# Autodesk Inventor assembly: GP5-100-TAV
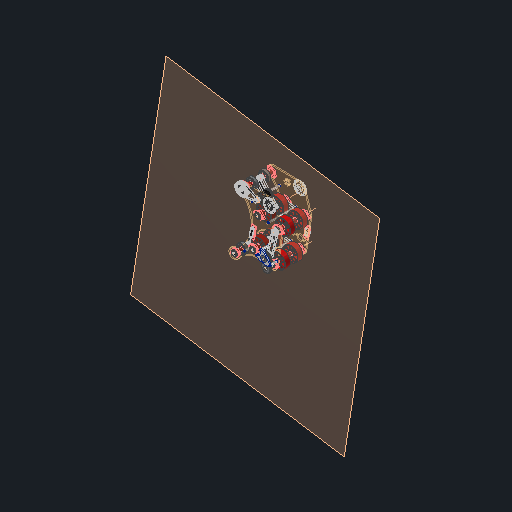
[picture p0: Inventor's stored thumbnail of the model, 512x512]
Saved by Autodesk Inventor 2023.4 (Build 274418000, 418)
## iProperties
Created: 2025-02-03
Part Number: GP5-100-TAV
Document SubType Name: Assembly
Designer: slick
Mass: 3623.08 g
Surface Area: 8652.96 cm^2
Volume: 1639.13 cm^3
Density: 2.21037 g/cm^3
Author: slick
## Documents named in this file (32)
- C:\Users\brand\OneDrive\Documents\GitHub\robotics 23\2025-ReefScape---CAD\Gripper\GP5\GP5-100-TAV.iam
- C:\Users\brand\OneDrive\Documents\GitHub\robotics 23\2025-ReefScape---CAD\Gripper\GP5\GP5-003.ipt
- C:\Users\brand\OneDrive\Documents\GitHub\robotics 23\2025-ReefScape---CAD\COMMON PARTS\BEARINGS\13_75mm_1_2_ThunderHex_ID_x_1_125_OD_x_0_313_WD_Flanged_Bearing_217-4006_MIR.ipt
- C:\Users\brand\OneDrive\Documents\GitHub\robotics 23\2025-ReefScape---CAD\Gripper\GP5\GP5-005.ipt
- C:\Users\brand\OneDrive\Documents\GitHub\robotics 23\2025-ReefScape---CAD\COMMON PARTS\WHEELS\2_OD_Straight_Flex_Wheel_217-6354.ipt
- C:\Users\brand\OneDrive\Documents\GitHub\robotics 23\2025-ReefScape---CAD\COMMON PARTS\WHEELS\am-3946 3IN 375Hex Compliant Wheel REV 3.ipt
- C:\Users\brand\OneDrive\Documents\GitHub\robotics 23\2025-ReefScape---CAD\COMMON PARTS\MOTORS\Minion.ipt
- C:\Users\brand\OneDrive\Documents\GitHub\robotics 23\2025-ReefScape---CAD\COMMON PARTS\PULLEYS\gt2\16T Gt2 Kracken PullyWCP-1178.ipt
- C:\Users\brand\OneDrive\Documents\GitHub\robotics 23\2025-ReefScape---CAD\COMMON PARTS\PULLEYS\gt2\60t_x_9mm_Wide_Double_Flange_Aluminum_Pulley_GT2_3mm_1_2_Hex_Bore_217-5876.ipt
- C:\Users\brand\OneDrive\Documents\GitHub\robotics 23\2025-ReefScape---CAD\COMMON PARTS\PULLEYS\gt2\24t_x_9mm_Wide_Double_Flange_Aluminum_Pulley_GT2_3mm_1_2_Hex_Bore_217-5875.ipt
- C:\Users\brand\OneDrive\Documents\GitHub\robotics 23\2025-ReefScape---CAD\COMMON PARTS\GEARS\20dp .5 hex\34t_Aluminum_Spur_Gear_20_DP_1_2_Hex_Bore_217-2706.ipt
- C:\Users\brand\OneDrive\Documents\GitHub\robotics 23\2025-ReefScape---CAD\Gripper\GP5\GP5-007.ipt
- C:\Users\brand\OneDrive\Documents\GitHub\robotics 23\2025-ReefScape---CAD\COMMON PARTS\BEARINGS\Bearing Retainer\Retainer.ipt
- C:\Users\brand\OneDrive\Documents\GitHub\robotics 23\2025-ReefScape---CAD\Gripper\GP5\GT2-100T.ipt
- C:\Users\brand\OneDrive\Documents\GitHub\robotics 23\2025-ReefScape---CAD\Gripper\GP5\GT2-90T.ipt
- C:\Users\brand\OneDrive\Documents\GitHub\robotics 23\2025-ReefScape---CAD\Gripper\GP5\GT2-90T16-60.ipt
- C:\Users\brand\OneDrive\Documents\GitHub\robotics 23\2025-ReefScape---CAD\Gripper\GP5\GT2-105T.ipt
- C:\Users\brand\OneDrive\Documents\GitHub\robotics 23\2025-ReefScape---CAD\Gripper\GP5\GP5-014.ipt
- C:\Users\brand\OneDrive\Documents\GitHub\robotics 23\2025-ReefScape---CAD\Gripper\GP5\GP5-019.ipt
- C:\Users\brand\OneDrive\Documents\GitHub\robotics 23\2025-ReefScape---CAD\COMMON PARTS\HUBS\WCP-1388.ipt
- C:\Users\brand\OneDrive\Documents\GitHub\robotics 23\2025-ReefScape---CAD\Gripper\GP5\GP5-023.ipt
- C:\Users\brand\OneDrive\Documents\GitHub\robotics 23\2025-ReefScape---CAD\Gripper\GP5\GP5-024.ipt
- C:\Users\brand\OneDrive\Documents\GitHub\robotics 23\2025-ReefScape---CAD\Gripper\GP5\GP5-025.ipt
- C:\Users\brand\OneDrive\Documents\GitHub\robotics 23\2025-ReefScape---CAD\Gripper\GP5\GP5-026.ipt
- C:\Users\brand\OneDrive\Documents\GitHub\robotics 23\2025-ReefScape---CAD\Gripper\GP5\GP5-013.ipt
- C:\Users\brand\OneDrive\Documents\GitHub\robotics 23\2025-ReefScape---CAD\Gripper\GP5\GP5-015.ipt
- C:\Users\brand\OneDrive\Documents\GitHub\robotics 23\2025-ReefScape---CAD\Gripper\GP5\GP5-016.ipt
- C:\Users\brand\OneDrive\Documents\GitHub\robotics 23\2025-ReefScape---CAD\Gripper\GP5\GP5-027.ipt
- C:\Users\brand\OneDrive\Documents\GitHub\robotics 23\2025-ReefScape---CAD\Gripper\GP5\GP5-028.ipt
- C:\Users\brand\OneDrive\Documents\GitHub\robotics 23\2025-ReefScape---CAD\Gripper\GP5\GP5-029.ipt
- C:\Users\brand\OneDrive\Documents\GitHub\robotics 23\2025-ReefScape---CAD\COMMON PARTS\BEARINGS\0_500_ID_x_1_125_OD_x_0_313_WD_Flanged_Bearing_217-2731.ipt
- C:\Users\brand\OneDrive\Documents\GitHub\robotics 23\2025-ReefScape---CAD\STEP files\sen36005_3d_model\With Flush Mount Spacer.iam
## Components (104 placed, 31 different names)
1. Minion:1 — Mate:18, Insert:15, Mate:19, Flush:1, Mate:22
2. 34t_Aluminum_Spur_Gear_20_DP_1_2_Hex_Bore_217-2706:1 — Mate:53, Flush:16, Mate:121
3. 34t_Aluminum_Spur_Gear_20_DP_1_2_Hex_Bore_217-2706:2 — Mate:51, Flush:16, Mate:56, Mate:72, Flush:78
4. WCP-1388:1 — Mate:80, Mate:81, Insert:54
5. WCP-1388:2 — Mate:79, Mate:81, Insert:53
6. GP5-026:1 — Insert:49, Insert:50
7. GP5-026:2 — Insert:45, Insert:46
8. GP5-026:3 — Insert:47, Insert:48
9. GP5-026:4 — Insert:51, Insert:52
10. GP5-014:3 — Mate:82, Mate:83
11. GP5-014:4 — Mate:84, Mate:85
12. GP5-015:1 — Mate:86, Mate:87
13. GP5-016:1 — Mate:88, Mate:89
14. GP5-016:2 — Mate:92, Mate:93
15. GP5-015:2 — Mate:97, Mate:100
16. GP5-015:3 — Mate:96, Mate:98
17. GP5-015:4 — Mate:95, Mate:99
18. GP5-013:2 — Mate:101, Mate:102
19. GP5-019:3 — Mate:104, Mate:105
20. GP5-019:4 — Mate:103, Mate:106
21. GP5-013:4 — Mate:108, Mate:109
22. GP5-013:5 — Mate:111, Mate:117
23. GP5-013:7 — Mate:113, Mate:116
24. GP5-027:1 — Insert:60, Insert:62, Insert:63, Mate:120
25. 0_500_ID_x_1_125_OD_x_0_313_WD_Flanged_Bearing_217-2731:1 — Insert:60, Mate:119, Flush:74, Mate:121
26. GP5-028:1 — Insert:62, Insert:64
27. GP5-028:2 — Insert:63, Insert:65
28. GP5-028:3 — Insert:58
29. GP5-029:1 — Mate:119, Flush:74
30. 0_500_ID_x_1_125_OD_x_0_313_WD_Flanged_Bearing_217-2731:2 — Insert:66
31. With Flush Mount Spacer:1 [sub-assembly] — Insert:69, Insert:70
32. With Flush Mount Spacer:2 [sub-assembly] — Insert:67, Insert:68
33. Retainer:13 — Insert:24, Insert:25
34. Retainer:12 — Insert:26, Insert:27
35. Retainer:11 — Insert:34, Insert:35
36. Retainer:10 — Insert:28, Insert:29
37. Retainer:9 — Insert:32, Insert:33
38. Retainer:8 — Insert:30, Insert:31
39. Retainer:7 — Insert:16, Insert:17
40. Retainer:6 — Insert:21, Insert:22
41. Retainer:5 — Insert:20, Insert:23
42. Retainer:4 — Insert:36, Insert:37, Insert:39
43. Retainer:3 — Insert:18, Insert:19
44. Retainer:1 — Insert:38, Insert:44
45. 13_75mm_1_2_ThunderHex_ID_x_1_125_OD_x_0_313_WD_Flanged_Bearing_217-4006_MIR:6 — Insert:9, Mate:13
46. 13_75mm_1_2_ThunderHex_ID_x_1_125_OD_x_0_313_WD_Flanged_Bearing_217-4006_MIR:14 — Insert:7, Mate:16, Mate:24
47. 13_75mm_1_2_ThunderHex_ID_x_1_125_OD_x_0_313_WD_Flanged_Bearing_217-4006_MIR:13 — Insert:8, Mate:12, Mate:64, Mate:66, Mate:67, Mate:69, Flush:73
48. 13_75mm_1_2_ThunderHex_ID_x_1_125_OD_x_0_313_WD_Flanged_Bearing_217-4006_MIR:12 — Insert:2
49. 13_75mm_1_2_ThunderHex_ID_x_1_125_OD_x_0_313_WD_Flanged_Bearing_217-4006_MIR:11 — Insert:6, Flush:82
50. 13_75mm_1_2_ThunderHex_ID_x_1_125_OD_x_0_313_WD_Flanged_Bearing_217-4006_MIR:10 — Insert:3, Flush:85
51. 13_75mm_1_2_ThunderHex_ID_x_1_125_OD_x_0_313_WD_Flanged_Bearing_217-4006_MIR:9 — Insert:5, Flush:83
52. 13_75mm_1_2_ThunderHex_ID_x_1_125_OD_x_0_313_WD_Flanged_Bearing_217-4006_MIR:8 — Insert:4
53. 13_75mm_1_2_ThunderHex_ID_x_1_125_OD_x_0_313_WD_Flanged_Bearing_217-4006_MIR:7 — Insert:1, Mate:28
54. 13_75mm_1_2_ThunderHex_ID_x_1_125_OD_x_0_313_WD_Flanged_Bearing_217-4006_MIR:5 — Insert:11, Mate:17, Mate:123
55. 13_75mm_1_2_ThunderHex_ID_x_1_125_OD_x_0_313_WD_Flanged_Bearing_217-4006_MIR:4 — Insert:10, Mate:14, Mate:26
56. 13_75mm_1_2_ThunderHex_ID_x_1_125_OD_x_0_313_WD_Flanged_Bearing_217-4006_MIR:3 — Insert:12, Mate:15, Mate:20, Mate:21
57. 24t_x_9mm_Wide_Double_Flange_Aluminum_Pulley_GT2_3mm_1_2_Hex_Bore_217-5875:7 — Mate:64, Mate:65
58. 24t_x_9mm_Wide_Double_Flange_Aluminum_Pulley_GT2_3mm_1_2_Hex_Bore_217-5875:8 — Mate:46, Flush:12
59. 24t_x_9mm_Wide_Double_Flange_Aluminum_Pulley_GT2_3mm_1_2_Hex_Bore_217-5875:9 — Mate:57, Mate:58, Mate:71
60. 24t_x_9mm_Wide_Double_Flange_Aluminum_Pulley_GT2_3mm_1_2_Hex_Bore_217-5875:10 — Mate:47, Mate:78, Flush:71, Flush:81, Flush:84
61. 24t_x_9mm_Wide_Double_Flange_Aluminum_Pulley_GT2_3mm_1_2_Hex_Bore_217-5875:12 — Mate:43, Mate:44, Flush:11, Flush:65, Mate:84
62. 24t_x_9mm_Wide_Double_Flange_Aluminum_Pulley_GT2_3mm_1_2_Hex_Bore_217-5875:13 — Mate:31, Mate:32, Flush:9, Mate:37, Mate:38, Mate:41
63. 24t_x_9mm_Wide_Double_Flange_Aluminum_Pulley_GT2_3mm_1_2_Hex_Bore_217-5875:14 — Mate:33, Mate:34, Flush:10, Mate:39
64. 24t_x_9mm_Wide_Double_Flange_Aluminum_Pulley_GT2_3mm_1_2_Hex_Bore_217-5875:15 — Mate:60, Mate:62, Flush:65, Flush:66, Flush:67
65. 24t_x_9mm_Wide_Double_Flange_Aluminum_Pulley_GT2_3mm_1_2_Hex_Bore_217-5875:16 — Mate:59, Mate:61, Mate:65, Flush:68
66. GT2-90T16-60:1 — Mate:22, Mate:23, Flush:2
67. GT2-105T:1 — Mate:52, Mate:54, Flush:77
68. GT2-100T:5 — Mate:69, Mate:70, Flush:68
69. GT2-90T:2 — Mate:71, Mate:72, Mate:73
70. GT2-90T:1 — Mate:77, Mate:78, Flush:71
71. GT2-100T:3 — Mate:67, Mate:68, Flush:67
72. GT2-100T:2 — Mate:36, Flush:10, Mate:44, Flush:11
73. GT2-100T:1 — Mate:35, Flush:9, Mate:45, Flush:12
74. 16T Gt2 Kracken PullyWCP-1178:1 — Mate:19, Flush:1
75. 60t_x_9mm_Wide_Double_Flange_Aluminum_Pulley_GT2_3mm_1_2_Hex_Bore_217-5876:1 — Mate:20, Mate:21, Mate:23, Flush:2, Flush:3
76. 24t_x_9mm_Wide_Double_Flange_Aluminum_Pulley_GT2_3mm_1_2_Hex_Bore_217-5875:1 — Mate:52, Mate:53, Flush:79, Mate:120
77. 24t_x_9mm_Wide_Double_Flange_Aluminum_Pulley_GT2_3mm_1_2_Hex_Bore_217-5875:2 — Mate:66, Flush:66, Mate:82
78. 24t_x_9mm_Wide_Double_Flange_Aluminum_Pulley_GT2_3mm_1_2_Hex_Bore_217-5875:4 — Mate:76, Mate:77, Flush:77, Flush:79, Mate:123
79. 24t_x_9mm_Wide_Double_Flange_Aluminum_Pulley_GT2_3mm_1_2_Hex_Bore_217-5875:5 — Mate:49, Flush:81, Mate:122
80. 24t_x_9mm_Wide_Double_Flange_Aluminum_Pulley_GT2_3mm_1_2_Hex_Bore_217-5875:6 — Mate:56, Mate:58, Mate:73, Flush:84
81. GP5-014:1 — Mate:32, Mate:33, Mate:35, Mate:36, Mate:38, Mate:39
82. GP5-014:2 — Mate:59, Mate:60, Mate:61, Mate:62, Mate:63
83. GP5-019:1 — Mate:31, Mate:37, Mate:42
84. GP5-019:2 — Mate:34, Mate:94
85. GP5-003:1 — Mate:1, Mate:2, Mate:3, Insert:1, Insert:2, Insert:3, Insert:4, Insert:5, Insert:6, Insert:16, Insert:17, Insert:18, Insert:19, Insert:20, Insert:21, Insert:22, Insert:23, Insert:36, Insert:37, Insert:38, Insert:39, Mate:80, Insert:44, Insert:46, Insert:47, Insert:50, Insert:51, Insert:53, Symmetry:1, Insert:69, Insert:70
86. GP5-003:2 — Mate:1, Mate:2, Mate:3, Insert:7, Insert:8, Insert:9, Insert:10, Insert:11, Insert:12, Mate:18, Insert:15, Mate:29, Insert:24, Insert:25, Insert:26, Insert:27, Insert:28, Insert:29, Insert:30, Insert:31, Insert:32, Insert:33, Insert:34, Insert:35, Mate:79, Insert:45, Insert:48, Insert:49, Insert:52, Insert:54, Insert:58, Insert:64, Insert:65, Insert:66, Symmetry:1, Insert:67, Insert:68
87. GP5-007:1 — Mate:15, Flush:3, Mate:87, Mate:97
88. GP5-025:1 — Mate:12, Mate:27, Flush:73, Mate:83, Mate:95, Mate:96, Mate:103, Mate:104
89. GP5-023:2 — Mate:11, Mate:13, Mate:57, Mate:63, Mate:68, Mate:70, Mate:108, Flush:85
90. GP5-023:1 — Mate:16, Mate:47, Mate:85, Mate:101, Flush:83
91. GP5-024:1 — Mate:14, Mate:51, Mate:92, Mate:111, Flush:78
92. GP5-005:6 — Mate:17, Mate:25, Mate:49, Mate:54, Mate:76, Mate:88, Mate:113, Flush:82
93. am-3946 3IN 375Hex Compliant Wheel REV 3:3 — Mate:26, Flush:5, Flush:6, Mate:117
94. am-3946 3IN 375Hex Compliant Wheel REV 3:2 — Mate:25, Flush:4, Flush:5, Mate:116
95. am-3946 3IN 375Hex Compliant Wheel REV 3:1 — Mate:24, Flush:4, Mate:43, Mate:102
96. am-3946 3IN 375Hex Compliant Wheel REV 3:4 — Mate:11, Flush:6, Flush:8, Mate:29, Mate:109
97. 2_OD_Straight_Flex_Wheel_217-6354:1 — Mate:28, Flush:7, Mate:94, Mate:100
98. 2_OD_Straight_Flex_Wheel_217-6354:2 — Mate:27, Flush:7, Flush:8, Mate:99, Mate:106
99. am-3946 3IN 375Hex Compliant Wheel REV 3:5 — Mate:93
100. am-3946 3IN 375Hex Compliant Wheel REV 3:6 — Mate:89, Mate:122
101. am-3946 3IN 375Hex Compliant Wheel REV 3:7 — Mate:45, Mate:46
102. am-3946 3IN 375Hex Compliant Wheel REV 3:8
103. 2_OD_Straight_Flex_Wheel_217-6354:3 — Mate:41, Mate:42, Mate:86
104. 2_OD_Straight_Flex_Wheel_217-6354:4 — Mate:98, Mate:105
## Component patterns: (2 elements, first: am-3946 3IN 375Hex Compliant Wheel REV 3:3 + am-3946 3IN 375Hex Compliant Wheel REV 3:2 + am-3946 3IN 375Hex Compliant Wheel REV 3:1 + am-3946 3IN 375Hex Compliant Wheel REV 3:4 + 2_OD_Straight_Flex_Wheel_217-6354:1 + 2_OD_Straight_Flex_Wheel_217-6354:2)
## Relationships (189: Mate 101, Insert 59, Flush 28, Symmetry 1)
- Mate:1: GP5-003:1 ↔ GP5-003:2
- Mate:2: GP5-003:1 ↔ GP5-003:2
- Mate:3 (139.7 mm): GP5-003:1 ↔ GP5-003:2
- Mate:11: GP5-023:2 ↔ am-3946 3IN 375Hex Compliant Wheel REV 3:4
- Insert:1: 13_75mm_1_2_ThunderHex_ID_x_1_125_OD_x_0_313_WD_Flanged_Bearing_217-4006_MIR:7 ↔ GP5-003:1
- Insert:2: 13_75mm_1_2_ThunderHex_ID_x_1_125_OD_x_0_313_WD_Flanged_Bearing_217-4006_MIR:12 ↔ GP5-003:1
- Insert:3: 13_75mm_1_2_ThunderHex_ID_x_1_125_OD_x_0_313_WD_Flanged_Bearing_217-4006_MIR:10 ↔ GP5-003:1
- Insert:4: 13_75mm_1_2_ThunderHex_ID_x_1_125_OD_x_0_313_WD_Flanged_Bearing_217-4006_MIR:8 ↔ GP5-003:1
- Insert:5: 13_75mm_1_2_ThunderHex_ID_x_1_125_OD_x_0_313_WD_Flanged_Bearing_217-4006_MIR:9 ↔ GP5-003:1
- Insert:6: 13_75mm_1_2_ThunderHex_ID_x_1_125_OD_x_0_313_WD_Flanged_Bearing_217-4006_MIR:11 ↔ GP5-003:1
- Insert:7: 13_75mm_1_2_ThunderHex_ID_x_1_125_OD_x_0_313_WD_Flanged_Bearing_217-4006_MIR:14 ↔ GP5-003:2
- Insert:8: 13_75mm_1_2_ThunderHex_ID_x_1_125_OD_x_0_313_WD_Flanged_Bearing_217-4006_MIR:13 ↔ GP5-003:2
- Insert:9: 13_75mm_1_2_ThunderHex_ID_x_1_125_OD_x_0_313_WD_Flanged_Bearing_217-4006_MIR:6 ↔ GP5-003:2
- Insert:10: 13_75mm_1_2_ThunderHex_ID_x_1_125_OD_x_0_313_WD_Flanged_Bearing_217-4006_MIR:4 ↔ GP5-003:2
- Insert:11: 13_75mm_1_2_ThunderHex_ID_x_1_125_OD_x_0_313_WD_Flanged_Bearing_217-4006_MIR:5 ↔ GP5-003:2
- Insert:12: 13_75mm_1_2_ThunderHex_ID_x_1_125_OD_x_0_313_WD_Flanged_Bearing_217-4006_MIR:3 ↔ GP5-003:2
- Mate:12: 13_75mm_1_2_ThunderHex_ID_x_1_125_OD_x_0_313_WD_Flanged_Bearing_217-4006_MIR:13 ↔ GP5-025:1
- Mate:13: 13_75mm_1_2_ThunderHex_ID_x_1_125_OD_x_0_313_WD_Flanged_Bearing_217-4006_MIR:6 ↔ GP5-023:2
- Mate:14: 13_75mm_1_2_ThunderHex_ID_x_1_125_OD_x_0_313_WD_Flanged_Bearing_217-4006_MIR:4 ↔ GP5-024:1
- Mate:15: 13_75mm_1_2_ThunderHex_ID_x_1_125_OD_x_0_313_WD_Flanged_Bearing_217-4006_MIR:3 ↔ GP5-007:1
- Mate:16: 13_75mm_1_2_ThunderHex_ID_x_1_125_OD_x_0_313_WD_Flanged_Bearing_217-4006_MIR:14 ↔ GP5-023:1
- Mate:17: 13_75mm_1_2_ThunderHex_ID_x_1_125_OD_x_0_313_WD_Flanged_Bearing_217-4006_MIR:5 ↔ GP5-005:6
- Mate:18: Minion:1 ↔ GP5-003:2
- Insert:15: Minion:1 ↔ GP5-003:2
- Mate:19: Minion:1 ↔ 16T Gt2 Kracken PullyWCP-1178:1
- Flush:1: Minion:1 ↔ 16T Gt2 Kracken PullyWCP-1178:1
- Mate:20: 13_75mm_1_2_ThunderHex_ID_x_1_125_OD_x_0_313_WD_Flanged_Bearing_217-4006_MIR:3 ↔ 60t_x_9mm_Wide_Double_Flange_Aluminum_Pulley_GT2_3mm_1_2_Hex_Bore_217-5876:1
- Mate:21: 13_75mm_1_2_ThunderHex_ID_x_1_125_OD_x_0_313_WD_Flanged_Bearing_217-4006_MIR:3 ↔ 60t_x_9mm_Wide_Double_Flange_Aluminum_Pulley_GT2_3mm_1_2_Hex_Bore_217-5876:1
- Mate:22: Minion:1 ↔ GT2-90T16-60:1
- Mate:23 (0.0762 mm): GT2-90T16-60:1 ↔ 60t_x_9mm_Wide_Double_Flange_Aluminum_Pulley_GT2_3mm_1_2_Hex_Bore_217-5876:1
- Flush:2: GT2-90T16-60:1 ↔ 60t_x_9mm_Wide_Double_Flange_Aluminum_Pulley_GT2_3mm_1_2_Hex_Bore_217-5876:1
- Flush:3: 60t_x_9mm_Wide_Double_Flange_Aluminum_Pulley_GT2_3mm_1_2_Hex_Bore_217-5876:1 ↔ GP5-007:1
- Mate:24: 13_75mm_1_2_ThunderHex_ID_x_1_125_OD_x_0_313_WD_Flanged_Bearing_217-4006_MIR:14 ↔ am-3946 3IN 375Hex Compliant Wheel REV 3:1
- Mate:25: GP5-005:6 ↔ am-3946 3IN 375Hex Compliant Wheel REV 3:2
- Mate:26: 13_75mm_1_2_ThunderHex_ID_x_1_125_OD_x_0_313_WD_Flanged_Bearing_217-4006_MIR:4 ↔ am-3946 3IN 375Hex Compliant Wheel REV 3:3
- Flush:4: am-3946 3IN 375Hex Compliant Wheel REV 3:2 ↔ am-3946 3IN 375Hex Compliant Wheel REV 3:1
- Flush:5: am-3946 3IN 375Hex Compliant Wheel REV 3:3 ↔ am-3946 3IN 375Hex Compliant Wheel REV 3:2
- Flush:6: am-3946 3IN 375Hex Compliant Wheel REV 3:3 ↔ am-3946 3IN 375Hex Compliant Wheel REV 3:4
- Mate:27: GP5-025:1 ↔ 2_OD_Straight_Flex_Wheel_217-6354:2
- Mate:28: 13_75mm_1_2_ThunderHex_ID_x_1_125_OD_x_0_313_WD_Flanged_Bearing_217-4006_MIR:7 ↔ 2_OD_Straight_Flex_Wheel_217-6354:1
- Flush:7: 2_OD_Straight_Flex_Wheel_217-6354:1 ↔ 2_OD_Straight_Flex_Wheel_217-6354:2
- Flush:8 (6.35 mm): am-3946 3IN 375Hex Compliant Wheel REV 3:4 ↔ 2_OD_Straight_Flex_Wheel_217-6354:2
- Mate:29 (25.4 mm): GP5-003:2 ↔ am-3946 3IN 375Hex Compliant Wheel REV 3:4
- Mate:31: 24t_x_9mm_Wide_Double_Flange_Aluminum_Pulley_GT2_3mm_1_2_Hex_Bore_217-5875:13 ↔ GP5-019:1
- Mate:32: 24t_x_9mm_Wide_Double_Flange_Aluminum_Pulley_GT2_3mm_1_2_Hex_Bore_217-5875:13 ↔ GP5-014:1
- Mate:33: 24t_x_9mm_Wide_Double_Flange_Aluminum_Pulley_GT2_3mm_1_2_Hex_Bore_217-5875:14 ↔ GP5-014:1
- Mate:34: 24t_x_9mm_Wide_Double_Flange_Aluminum_Pulley_GT2_3mm_1_2_Hex_Bore_217-5875:14 ↔ GP5-019:2
- Mate:35: GT2-100T:1 ↔ GP5-014:1
- Mate:36: GT2-100T:2 ↔ GP5-014:1
- Flush:9: 24t_x_9mm_Wide_Double_Flange_Aluminum_Pulley_GT2_3mm_1_2_Hex_Bore_217-5875:13 ↔ GT2-100T:1
- Flush:10: 24t_x_9mm_Wide_Double_Flange_Aluminum_Pulley_GT2_3mm_1_2_Hex_Bore_217-5875:14 ↔ GT2-100T:2
- Mate:37: 24t_x_9mm_Wide_Double_Flange_Aluminum_Pulley_GT2_3mm_1_2_Hex_Bore_217-5875:13 ↔ GP5-019:1
- Mate:38: 24t_x_9mm_Wide_Double_Flange_Aluminum_Pulley_GT2_3mm_1_2_Hex_Bore_217-5875:13 ↔ GP5-014:1
- Mate:39: 24t_x_9mm_Wide_Double_Flange_Aluminum_Pulley_GT2_3mm_1_2_Hex_Bore_217-5875:14 ↔ GP5-014:1
- Mate:41: 24t_x_9mm_Wide_Double_Flange_Aluminum_Pulley_GT2_3mm_1_2_Hex_Bore_217-5875:13 ↔ 2_OD_Straight_Flex_Wheel_217-6354:3
- Mate:42: GP5-019:1 ↔ 2_OD_Straight_Flex_Wheel_217-6354:3
- Insert:16: Retainer:7 ↔ GP5-003:1
- Insert:17: Retainer:7 ↔ GP5-003:1
- Insert:18: Retainer:3 ↔ GP5-003:1
- Insert:19: Retainer:3 ↔ GP5-003:1
- Insert:20: Retainer:5 ↔ GP5-003:1
- Insert:21: Retainer:6 ↔ GP5-003:1
- Insert:22: Retainer:6 ↔ GP5-003:1
- Insert:23: Retainer:5 ↔ GP5-003:1
- Insert:24: Retainer:13 ↔ GP5-003:2
- Insert:25: Retainer:13 ↔ GP5-003:2
- Insert:26: Retainer:12 ↔ GP5-003:2
- Insert:27: Retainer:12 ↔ GP5-003:2
- Insert:28: Retainer:10 ↔ GP5-003:2
- Insert:29: Retainer:10 ↔ GP5-003:2
- Insert:30: Retainer:8 ↔ GP5-003:2
- Insert:31: Retainer:8 ↔ GP5-003:2
- Insert:32: Retainer:9 ↔ GP5-003:2
- Insert:33: Retainer:9 ↔ GP5-003:2
- Insert:34: Retainer:11 ↔ GP5-003:2
- Insert:35: Retainer:11 ↔ GP5-003:2
- Insert:36: Retainer:4 ↔ GP5-003:1
- Insert:37: Retainer:4 ↔ GP5-003:1
- Insert:38: Retainer:1 ↔ GP5-003:1
- Insert:39: Retainer:4 ↔ GP5-003:1
- Mate:43: 24t_x_9mm_Wide_Double_Flange_Aluminum_Pulley_GT2_3mm_1_2_Hex_Bore_217-5875:12 ↔ am-3946 3IN 375Hex Compliant Wheel REV 3:1
- Mate:44 (0.0762 mm): 24t_x_9mm_Wide_Double_Flange_Aluminum_Pulley_GT2_3mm_1_2_Hex_Bore_217-5875:12 ↔ GT2-100T:2
- Flush:11: 24t_x_9mm_Wide_Double_Flange_Aluminum_Pulley_GT2_3mm_1_2_Hex_Bore_217-5875:12 ↔ GT2-100T:2
- Mate:45 (0.0762 mm): GT2-100T:1 ↔ am-3946 3IN 375Hex Compliant Wheel REV 3:7
- Mate:46: 24t_x_9mm_Wide_Double_Flange_Aluminum_Pulley_GT2_3mm_1_2_Hex_Bore_217-5875:8 ↔ am-3946 3IN 375Hex Compliant Wheel REV 3:7
- Flush:12: 24t_x_9mm_Wide_Double_Flange_Aluminum_Pulley_GT2_3mm_1_2_Hex_Bore_217-5875:8 ↔ GT2-100T:1
- Mate:47: 24t_x_9mm_Wide_Double_Flange_Aluminum_Pulley_GT2_3mm_1_2_Hex_Bore_217-5875:10 ↔ GP5-023:1
- Mate:49: 24t_x_9mm_Wide_Double_Flange_Aluminum_Pulley_GT2_3mm_1_2_Hex_Bore_217-5875:5 ↔ GP5-005:6
- Mate:51: 34t_Aluminum_Spur_Gear_20_DP_1_2_Hex_Bore_217-2706:2 ↔ GP5-024:1
- Mate:52: GT2-105T:1 ↔ 24t_x_9mm_Wide_Double_Flange_Aluminum_Pulley_GT2_3mm_1_2_Hex_Bore_217-5875:1
- Mate:53: 34t_Aluminum_Spur_Gear_20_DP_1_2_Hex_Bore_217-2706:1 ↔ 24t_x_9mm_Wide_Double_Flange_Aluminum_Pulley_GT2_3mm_1_2_Hex_Bore_217-5875:1
- Flush:16: 34t_Aluminum_Spur_Gear_20_DP_1_2_Hex_Bore_217-2706:1 ↔ 34t_Aluminum_Spur_Gear_20_DP_1_2_Hex_Bore_217-2706:2
- Mate:54 (0.0762 mm): GT2-105T:1 ↔ GP5-005:6
- Mate:56: 34t_Aluminum_Spur_Gear_20_DP_1_2_Hex_Bore_217-2706:2 ↔ 24t_x_9mm_Wide_Double_Flange_Aluminum_Pulley_GT2_3mm_1_2_Hex_Bore_217-5875:6
- Mate:57: 24t_x_9mm_Wide_Double_Flange_Aluminum_Pulley_GT2_3mm_1_2_Hex_Bore_217-5875:9 ↔ GP5-023:2
- Mate:58: 24t_x_9mm_Wide_Double_Flange_Aluminum_Pulley_GT2_3mm_1_2_Hex_Bore_217-5875:9 ↔ 24t_x_9mm_Wide_Double_Flange_Aluminum_Pulley_GT2_3mm_1_2_Hex_Bore_217-5875:6
- Mate:59: 24t_x_9mm_Wide_Double_Flange_Aluminum_Pulley_GT2_3mm_1_2_Hex_Bore_217-5875:16 ↔ GP5-014:2
- Mate:60: 24t_x_9mm_Wide_Double_Flange_Aluminum_Pulley_GT2_3mm_1_2_Hex_Bore_217-5875:15 ↔ GP5-014:2
- Mate:61: 24t_x_9mm_Wide_Double_Flange_Aluminum_Pulley_GT2_3mm_1_2_Hex_Bore_217-5875:16 ↔ GP5-014:2
- Mate:62: 24t_x_9mm_Wide_Double_Flange_Aluminum_Pulley_GT2_3mm_1_2_Hex_Bore_217-5875:15 ↔ GP5-014:2
- Mate:63: GP5-014:2 ↔ GP5-023:2
- Flush:65: 24t_x_9mm_Wide_Double_Flange_Aluminum_Pulley_GT2_3mm_1_2_Hex_Bore_217-5875:12 ↔ 24t_x_9mm_Wide_Double_Flange_Aluminum_Pulley_GT2_3mm_1_2_Hex_Bore_217-5875:15
- Mate:64: 13_75mm_1_2_ThunderHex_ID_x_1_125_OD_x_0_313_WD_Flanged_Bearing_217-4006_MIR:13 ↔ 24t_x_9mm_Wide_Double_Flange_Aluminum_Pulley_GT2_3mm_1_2_Hex_Bore_217-5875:7
- Mate:65: 24t_x_9mm_Wide_Double_Flange_Aluminum_Pulley_GT2_3mm_1_2_Hex_Bore_217-5875:7 ↔ 24t_x_9mm_Wide_Double_Flange_Aluminum_Pulley_GT2_3mm_1_2_Hex_Bore_217-5875:16
- Mate:66: 13_75mm_1_2_ThunderHex_ID_x_1_125_OD_x_0_313_WD_Flanged_Bearing_217-4006_MIR:13 ↔ 24t_x_9mm_Wide_Double_Flange_Aluminum_Pulley_GT2_3mm_1_2_Hex_Bore_217-5875:2
- Flush:66: 24t_x_9mm_Wide_Double_Flange_Aluminum_Pulley_GT2_3mm_1_2_Hex_Bore_217-5875:15 ↔ 24t_x_9mm_Wide_Double_Flange_Aluminum_Pulley_GT2_3mm_1_2_Hex_Bore_217-5875:2
- Mate:67: 13_75mm_1_2_ThunderHex_ID_x_1_125_OD_x_0_313_WD_Flanged_Bearing_217-4006_MIR:13 ↔ GT2-100T:3
- Mate:68 (0.0508 mm): GT2-100T:3 ↔ GP5-023:2
- Flush:67: 24t_x_9mm_Wide_Double_Flange_Aluminum_Pulley_GT2_3mm_1_2_Hex_Bore_217-5875:15 ↔ GT2-100T:3
- Mate:69: 13_75mm_1_2_ThunderHex_ID_x_1_125_OD_x_0_313_WD_Flanged_Bearing_217-4006_MIR:13 ↔ GT2-100T:5
- Mate:70 (0.0508 mm): GT2-100T:5 ↔ GP5-023:2
- Flush:68: 24t_x_9mm_Wide_Double_Flange_Aluminum_Pulley_GT2_3mm_1_2_Hex_Bore_217-5875:16 ↔ GT2-100T:5
- Mate:71: 24t_x_9mm_Wide_Double_Flange_Aluminum_Pulley_GT2_3mm_1_2_Hex_Bore_217-5875:9 ↔ GT2-90T:2
- Mate:72 (0.0508 mm): 34t_Aluminum_Spur_Gear_20_DP_1_2_Hex_Bore_217-2706:2 ↔ GT2-90T:2
- Mate:73: GT2-90T:2 ↔ 24t_x_9mm_Wide_Double_Flange_Aluminum_Pulley_GT2_3mm_1_2_Hex_Bore_217-5875:6
- Mate:76: 24t_x_9mm_Wide_Double_Flange_Aluminum_Pulley_GT2_3mm_1_2_Hex_Bore_217-5875:4 ↔ GP5-005:6
- Mate:77: GT2-90T:1 ↔ 24t_x_9mm_Wide_Double_Flange_Aluminum_Pulley_GT2_3mm_1_2_Hex_Bore_217-5875:4
- Mate:78 (0.0508 mm): 24t_x_9mm_Wide_Double_Flange_Aluminum_Pulley_GT2_3mm_1_2_Hex_Bore_217-5875:10 ↔ GT2-90T:1
- Flush:71: 24t_x_9mm_Wide_Double_Flange_Aluminum_Pulley_GT2_3mm_1_2_Hex_Bore_217-5875:10 ↔ GT2-90T:1
- Flush:73: 13_75mm_1_2_ThunderHex_ID_x_1_125_OD_x_0_313_WD_Flanged_Bearing_217-4006_MIR:13 ↔ GP5-025:1
- Mate:79: WCP-1388:2 ↔ GP5-003:2
- Mate:80: WCP-1388:1 ↔ GP5-003:1
- Mate:81: WCP-1388:1 ↔ WCP-1388:2
- Insert:44: Retainer:1 ↔ GP5-003:1
- Insert:45: GP5-026:2 ↔ GP5-003:2
- Insert:46: GP5-026:2 ↔ GP5-003:1
- Insert:47: GP5-026:3 ↔ GP5-003:1
- Insert:48: GP5-026:3 ↔ GP5-003:2
- Insert:49: GP5-026:1 ↔ GP5-003:2
- Insert:50: GP5-026:1 ↔ GP5-003:1
- Insert:51: GP5-026:4 ↔ GP5-003:1
- Insert:52: GP5-026:4 ↔ GP5-003:2
- Mate:82: GP5-014:3 ↔ 24t_x_9mm_Wide_Double_Flange_Aluminum_Pulley_GT2_3mm_1_2_Hex_Bore_217-5875:2
- Mate:83: GP5-014:3 ↔ GP5-025:1
- Mate:84: GP5-014:4 ↔ 24t_x_9mm_Wide_Double_Flange_Aluminum_Pulley_GT2_3mm_1_2_Hex_Bore_217-5875:12
- Mate:85: GP5-014:4 ↔ GP5-023:1
- Mate:86: GP5-015:1 ↔ 2_OD_Straight_Flex_Wheel_217-6354:3
- Mate:87: GP5-015:1 ↔ GP5-007:1
- Mate:88: GP5-016:1 ↔ GP5-005:6
- Mate:89: GP5-016:1 ↔ am-3946 3IN 375Hex Compliant Wheel REV 3:6
- Mate:92: GP5-016:2 ↔ GP5-024:1
- Mate:93: GP5-016:2 ↔ am-3946 3IN 375Hex Compliant Wheel REV 3:5
- Mate:94: GP5-019:2 ↔ 2_OD_Straight_Flex_Wheel_217-6354:1
- Mate:95: GP5-015:4 ↔ GP5-025:1
- Mate:96: GP5-015:3 ↔ GP5-025:1
- Mate:97: GP5-015:2 ↔ GP5-007:1
- Insert:53: WCP-1388:2 ↔ GP5-003:1
- Insert:54: WCP-1388:1 ↔ GP5-003:2
- Mate:98: GP5-015:3 ↔ 2_OD_Straight_Flex_Wheel_217-6354:4
- Mate:99: GP5-015:4 ↔ 2_OD_Straight_Flex_Wheel_217-6354:2
- Mate:100: GP5-015:2 ↔ 2_OD_Straight_Flex_Wheel_217-6354:1
- Mate:101: GP5-013:2 ↔ GP5-023:1
- Mate:102: GP5-013:2 ↔ am-3946 3IN 375Hex Compliant Wheel REV 3:1
- Mate:103: GP5-019:4 ↔ GP5-025:1
- Mate:104: GP5-019:3 ↔ GP5-025:1
- Mate:105: GP5-019:3 ↔ 2_OD_Straight_Flex_Wheel_217-6354:4
- Mate:106: GP5-019:4 ↔ 2_OD_Straight_Flex_Wheel_217-6354:2
- Mate:108: GP5-013:4 ↔ GP5-023:2
- Mate:109: GP5-013:4 ↔ am-3946 3IN 375Hex Compliant Wheel REV 3:4
- Mate:111: GP5-013:5 ↔ GP5-024:1
- Mate:113: GP5-013:7 ↔ GP5-005:6
- Mate:116: GP5-013:7 ↔ am-3946 3IN 375Hex Compliant Wheel REV 3:2
- Mate:117: GP5-013:5 ↔ am-3946 3IN 375Hex Compliant Wheel REV 3:3
- Insert:58: GP5-028:3 ↔ GP5-003:2
- Insert:60: GP5-027:1 ↔ 0_500_ID_x_1_125_OD_x_0_313_WD_Flanged_Bearing_217-2731:1
- Insert:62: GP5-027:1 ↔ GP5-028:1
- Insert:63: GP5-027:1 ↔ GP5-028:2
- Insert:64: GP5-028:1 ↔ GP5-003:2
- Insert:65: GP5-028:2 ↔ GP5-003:2
- Insert:66: 0_500_ID_x_1_125_OD_x_0_313_WD_Flanged_Bearing_217-2731:2 ↔ GP5-003:2
- Mate:119: 0_500_ID_x_1_125_OD_x_0_313_WD_Flanged_Bearing_217-2731:1 ↔ GP5-029:1
- Flush:74: 0_500_ID_x_1_125_OD_x_0_313_WD_Flanged_Bearing_217-2731:1 ↔ GP5-029:1
- Flush:77: GT2-105T:1 ↔ 24t_x_9mm_Wide_Double_Flange_Aluminum_Pulley_GT2_3mm_1_2_Hex_Bore_217-5875:4
- Flush:78: 34t_Aluminum_Spur_Gear_20_DP_1_2_Hex_Bore_217-2706:2 ↔ GP5-024:1
- Flush:79: 24t_x_9mm_Wide_Double_Flange_Aluminum_Pulley_GT2_3mm_1_2_Hex_Bore_217-5875:1 ↔ 24t_x_9mm_Wide_Double_Flange_Aluminum_Pulley_GT2_3mm_1_2_Hex_Bore_217-5875:4
- Mate:120: GP5-027:1 ↔ 24t_x_9mm_Wide_Double_Flange_Aluminum_Pulley_GT2_3mm_1_2_Hex_Bore_217-5875:1
- Mate:121: 34t_Aluminum_Spur_Gear_20_DP_1_2_Hex_Bore_217-2706:1 ↔ 0_500_ID_x_1_125_OD_x_0_313_WD_Flanged_Bearing_217-2731:1
- Flush:81: 24t_x_9mm_Wide_Double_Flange_Aluminum_Pulley_GT2_3mm_1_2_Hex_Bore_217-5875:10 ↔ 24t_x_9mm_Wide_Double_Flange_Aluminum_Pulley_GT2_3mm_1_2_Hex_Bore_217-5875:5
- Mate:122 (1.5875 mm): 24t_x_9mm_Wide_Double_Flange_Aluminum_Pulley_GT2_3mm_1_2_Hex_Bore_217-5875:5 ↔ am-3946 3IN 375Hex Compliant Wheel REV 3:6
- Flush:82: 13_75mm_1_2_ThunderHex_ID_x_1_125_OD_x_0_313_WD_Flanged_Bearing_217-4006_MIR:11 ↔ GP5-005:6
- Flush:83: 13_75mm_1_2_ThunderHex_ID_x_1_125_OD_x_0_313_WD_Flanged_Bearing_217-4006_MIR:9 ↔ GP5-023:1
- Mate:123: 13_75mm_1_2_ThunderHex_ID_x_1_125_OD_x_0_313_WD_Flanged_Bearing_217-4006_MIR:5 ↔ 24t_x_9mm_Wide_Double_Flange_Aluminum_Pulley_GT2_3mm_1_2_Hex_Bore_217-5875:4
- Flush:84: 24t_x_9mm_Wide_Double_Flange_Aluminum_Pulley_GT2_3mm_1_2_Hex_Bore_217-5875:10 ↔ 24t_x_9mm_Wide_Double_Flange_Aluminum_Pulley_GT2_3mm_1_2_Hex_Bore_217-5875:6
- Flush:85: 13_75mm_1_2_ThunderHex_ID_x_1_125_OD_x_0_313_WD_Flanged_Bearing_217-4006_MIR:10 ↔ GP5-023:2
- Symmetry:1: GP5-003:1 ↔ GP5-003:2
- Insert:67: With Flush Mount Spacer:2 ↔ GP5-003:2
- Insert:68: With Flush Mount Spacer:2 ↔ GP5-003:2
- Insert:69: With Flush Mount Spacer:1 ↔ GP5-003:1
- Insert:70: With Flush Mount Spacer:1 ↔ GP5-003:1
